# Autodesk Inventor assembly: Hex Shaft Assembly
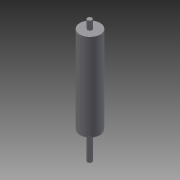
[picture p0: Inventor's stored thumbnail of the model, 180x180]
Saved by Autodesk Inventor 2015 (Build 190159000, 159)
## iProperties
Created: 2015-02-04
Part Number: Hex Shaft Assembly
Document SubType Name: Assembly
Designer: kaurdha17
Author: kaurdha17
## Documents named in this file (4)
- H:\Hex Shaft Assembly.iam
- H:\Hex Plug.ipt
- H:\PVC Pipe.ipt
- H:\Hex Shaft.ipt
## Components (4 placed, 3 different names)
1. Hex Plug:1 — Insert:1, Flush:1, Mate:1
2. PVC Pipe:1 — Insert:1, Insert:2
3. Hex Shaft:1 — Flush:1, Mate:1
4. Hex Plug:2 — Insert:2
## Relationships (4: Insert 2, Flush 1, Mate 1)
- Insert:1: Hex Plug:1 ↔ PVC Pipe:1
- Flush:1 (-25.4 mm): Hex Plug:1 ↔ Hex Shaft:1
- Mate:1: Hex Plug:1 ↔ Hex Shaft:1
- Insert:2: PVC Pipe:1 ↔ Hex Plug:2
